# Autodesk Inventor assembly: assembly
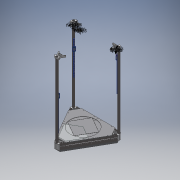
[picture p0: Inventor's stored thumbnail of the model, 180x180]
Saved by Autodesk Inventor 2016 SP1 (Build 200210100, 210)
## iProperties
Created: 2016-04-14
Part Number: assembly
Document SubType Name: Assembly
Designer: ubik
Author: ubik
## Documents named in this file (15)
- E:\GitHub\kossel-XXL\assembly.iam
- E:\GitHub\kossel-XXL\vertex\vertex-bottom.ipt
- E:\GitHub\kossel-XXL\vertex.ipt
- E:\GitHub\kossel-XXL\20x20\20x20-500.ipt
- E:\GitHub\kossel-XXL\20x20.ipt
- E:\GitHub\kossel-XXL\bottom plate.ipt
- E:\GitHub\kossel-XXL\bottom half.ipt
- E:\GitHub\kossel-XXL\alu plate.ipt
- E:\GitHub\kossel-XXL\bottom top plate.ipt
- E:\GitHub\kossel-XXL\heated bed.ipt
- E:\GitHub\kossel-XXL\20x20\20x20-950.ipt
- E:\GitHub\kossel-XXL\Linear Rail.ipt
- E:\GitHub\kossel-XXL\vertex\vertex-top.ipt
- E:\GitHub\kossel-XXL\Carriage.ipt
- E:\GitHub\kossel-XXL\assembly endstop.iam
## Components (31 placed, 12 different names)
1. vertex-bottom:1 — Flush:1, Mate:1, Mate:2, Mate:3, Flush:2, Mate:4, Mate:6, Flush:5, Flush:6, Mate:7, Flush:7, Mate:8, Mate:9, Mate:18, Mate:19, Flush:17
2. 20x20-500:1 — Mate:3, Flush:2, Mate:4
3. 20x20-500:2 — Flush:1, Mate:1, Mate:2, Mate:5, Flush:3, Mate:13
4. vertex-bottom:2 — Mate:5, Flush:3, Mate:13, Mate:14, Mate:15, Flush:10, Mate:16, Flush:12, Flush:18, Mate:20, Mate:21
5. vertex-bottom:3 — Mate:10, Flush:8, Mate:11, Mate:12, Flush:11, Flush:15, Mate:22, Mate:23, Flush:19
6. 20x20-500:3 — Flush:7, Mate:8, Mate:9
7. 20x20-500:4 — Mate:6, Flush:5, Flush:6, Mate:7, Mate:10, Flush:8, Mate:11, Mate:17
8. 20x20-500:5 — Mate:14, Mate:15, Flush:10
9. 20x20-500:6 — Mate:12, Flush:11, Mate:16
10. bottom plate:1 — Flush:12, Flush:13
11. bottom half:1 — Flush:13
12. alu plate:1 — Mate:17
13. heated bed:1 — Flush:16
14. 20x20-950:7 — Flush:18, Mate:20, Mate:21, Mate:26, Flush:22, Mate:29, Mate:30, Flush:24, Mate:43, Mate:44
15. 20x20-950:8 — Mate:22, Mate:23, Flush:19, Mate:24, Flush:20, Flush:23, Mate:27, Mate:28, Mate:39, Mate:40
16. 20x20-950:9 — Mate:18, Mate:19, Flush:17, Mate:25, Flush:21, Mate:31, Mate:32, Flush:25
17. Linear Rail:1 — Mate:24, Flush:20, Mate:33, Mate:34
18. Linear Rail:2 — Mate:25, Flush:21, Mate:37, Mate:38
19. Linear Rail:3 — Mate:26, Flush:22, Mate:35, Mate:36
20. vertex-top:4 — Mate:31, Mate:32, Flush:25
21. vertex-top:5 — Mate:29, Mate:30, Flush:24, Mate:42
22. vertex-top:6 — Flush:23, Mate:27, Mate:28, Mate:41
23. Carriage:1 — Mate:33, Mate:34
24. Carriage:2 — Mate:37, Mate:38
25. Carriage:3 — Mate:35, Mate:36
26. assembly endstop:1 [sub-assembly]
27. assembly endstop:2 [sub-assembly] — Mate:39, Mate:40, Mate:41
28. assembly endstop:3 [sub-assembly] — Mate:42, Mate:43, Mate:44
29. bottom top plate:1 — Flush:15, Flush:16
30. bottom top plate:2
31. bottom top plate:3
## Component patterns: (3 elements, first: bottom top plate:1)
## Relationships (66: Mate 44, Flush 22)
- Flush:1: vertex-bottom:1 ↔ 20x20-500:2
- Mate:1: vertex-bottom:1 ↔ 20x20-500:2
- Mate:2: vertex-bottom:1 ↔ 20x20-500:2
- Mate:3: vertex-bottom:1 ↔ 20x20-500:1
- Flush:2: vertex-bottom:1 ↔ 20x20-500:1
- Mate:4: vertex-bottom:1 ↔ 20x20-500:1
- Mate:5: 20x20-500:2 ↔ vertex-bottom:2
- Flush:3: 20x20-500:2 ↔ vertex-bottom:2
- Mate:6: vertex-bottom:1 ↔ 20x20-500:4
- Flush:5: vertex-bottom:1 ↔ 20x20-500:4
- Flush:6: vertex-bottom:1 ↔ 20x20-500:4
- Mate:7: vertex-bottom:1 ↔ 20x20-500:4
- Flush:7: vertex-bottom:1 ↔ 20x20-500:3
- Mate:8: vertex-bottom:1 ↔ 20x20-500:3
- Mate:9: vertex-bottom:1 ↔ 20x20-500:3
- Mate:10: vertex-bottom:3 ↔ 20x20-500:4
- Flush:8: vertex-bottom:3 ↔ 20x20-500:4
- Mate:11: vertex-bottom:3 ↔ 20x20-500:4
- Mate:12: vertex-bottom:3 ↔ 20x20-500:6
- Mate:13: 20x20-500:2 ↔ vertex-bottom:2
- Mate:14: vertex-bottom:2 ↔ 20x20-500:5
- Mate:15: vertex-bottom:2 ↔ 20x20-500:5
- Flush:10: vertex-bottom:2 ↔ 20x20-500:5
- Flush:11: vertex-bottom:3 ↔ 20x20-500:6
- Mate:16: vertex-bottom:2 ↔ 20x20-500:6
- Flush:12: vertex-bottom:2 ↔ bottom plate:1
- Flush:13: bottom plate:1 ↔ bottom half:1
- Flush:15: vertex-bottom:3 ↔ bottom top plate:1
- Mate:17 (8 mm): 20x20-500:4 ↔ alu plate:1
- Flush:16: heated bed:1 ↔ bottom top plate:1
- Mate:18: vertex-bottom:1 ↔ 20x20-950:9
- Mate:19: vertex-bottom:1 ↔ 20x20-950:9
- Flush:17: vertex-bottom:1 ↔ 20x20-950:9
- Flush:18: vertex-bottom:2 ↔ 20x20-950:7
- Mate:20: vertex-bottom:2 ↔ 20x20-950:7
- Mate:21: vertex-bottom:2 ↔ 20x20-950:7
- Mate:22: vertex-bottom:3 ↔ 20x20-950:8
- Mate:23: vertex-bottom:3 ↔ 20x20-950:8
- Flush:19: vertex-bottom:3 ↔ 20x20-950:8
- Mate:24: 20x20-950:8 ↔ Linear Rail:1
- Flush:20 (-4 mm): 20x20-950:8 ↔ Linear Rail:1
- Mate:25: 20x20-950:9 ↔ Linear Rail:2
- Flush:21 (4 mm): 20x20-950:9 ↔ Linear Rail:2
- Mate:26: 20x20-950:7 ↔ Linear Rail:3
- Flush:22 (-4 mm): 20x20-950:7 ↔ Linear Rail:3
- Flush:23: 20x20-950:8 ↔ vertex-top:6
- Mate:27: 20x20-950:8 ↔ vertex-top:6
- Mate:28: 20x20-950:8 ↔ vertex-top:6
- Mate:29: 20x20-950:7 ↔ vertex-top:5
- Mate:30: 20x20-950:7 ↔ vertex-top:5
- Flush:24: 20x20-950:7 ↔ vertex-top:5
- Mate:31: 20x20-950:9 ↔ vertex-top:4
- Mate:32: 20x20-950:9 ↔ vertex-top:4
- Flush:25: 20x20-950:9 ↔ vertex-top:4
- Mate:33 (0.5 mm): Linear Rail:1 ↔ Carriage:1
- Mate:34 (0.5 mm): Linear Rail:1 ↔ Carriage:1
- Mate:35 (0.5 mm): Linear Rail:3 ↔ Carriage:3
- Mate:36 (0.5 mm): Linear Rail:3 ↔ Carriage:3
- Mate:37 (0.5 mm): Linear Rail:2 ↔ Carriage:2
- Mate:38 (0.5 mm): Linear Rail:2 ↔ Carriage:2
- Mate:39: 20x20-950:8 ↔ assembly endstop:2
- Mate:40 (-10 mm): 20x20-950:8 ↔ assembly endstop:2
- Mate:41: vertex-top:6 ↔ assembly endstop:2
- Mate:42: vertex-top:5 ↔ assembly endstop:3
- Mate:43: 20x20-950:7 ↔ assembly endstop:3
- Mate:44 (-10 mm): 20x20-950:7 ↔ assembly endstop:3
